# Autodesk Inventor assembly: BoxBeamDBAssembly
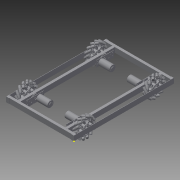
[picture p0: Inventor's stored thumbnail of the model, 180x180]
Saved by Autodesk Inventor 2015 (Build 190159000, 159)
## iProperties
Created: 2015-01-14
Part Number: BoxBeamDBAssembly
Document SubType Name: Assembly
Designer: chapale16
Author: chapale16
## Documents named in this file (13)
- \\lhssvr02\Homedirs\Robotics Club\CAD Model 2015\CDR prep\BoxBeamDBAssembly.iam
- \\lhssvr02\Homedirs\Robotics Club\CAD Model 2015\CDR prep\Frame front-back.ipt
- \\lhssvr02\Homedirs\Robotics Club\CAD Model 2015\CDR prep\Frame sides.ipt
- \\lhssvr02\Homedirs\Robotics Club\CAD Model 2015\Parts Folder\Wheels\Right Vex Mec Wheel.iam
- \\lhssvr02\Homedirs\Robotics Club\CAD Model 2015\Parts Folder\Gear Boxes\CIMple Box with motors.iam
- \\lhssvr02\Homedirs\Robotics Club\CAD Model 2015\CDR prep\Bumpers.ipt
- \\lhssvr02\Homedirs\Robotics Club\CAD Model 2015\GearBox Assembly_MIR.iam
- \\lhssvr02\Homedirs\Robotics Club\CAD Model 2015\Parts Folder\Wheels\Right Vex Mec Wheel_MIR.iam
- \\lhssvr02\Homedirs\Robotics Club\CAD Model 2015\GearBox Assembly_MIR_MIR.iam
- \\lhssvr02\Homedirs\Robotics Club\CAD Model 2015\Parts Folder\Wheels\Right Vex Mec Wheel_MIR1.iam
- \\lhssvr02\Homedirs\Robotics Club\CAD Model 2015\GearBox Assembly_MIR_MIR1.iam
- \\lhssvr02\Homedirs\Robotics Club\CAD Model 2015\Parts Folder\Wheels\Right Vex Mec Wheel_MIR_MIR.iam
- \\lhssvr02\Homedirs\Robotics Club\CAD Model 2015\GearBox Assembly_MIR_MIR_MIR.iam
## Components (18 placed, 12 different names)
1. Frame front-back:1 — Mate:3, Flush:5, Flush:6, Flush:7, Mate:4, Mate:5, Flush:8, Symmetry:1
2. Frame front-back:2 — Mate:1, Flush:1, Flush:2, Mate:2, Flush:3, Flush:4, Mate:6, Flush:9, Mate:7, Symmetry:1
3. Frame sides:1 — Mate:1, Flush:1, Flush:2, Mate:3, Flush:5, Flush:6, Mate:8, Mate:9, Mate:10, Symmetry:2
4. Frame sides:2 — Mate:2, Flush:3, Flush:4, Flush:7, Symmetry:2
5. Right Vex Mec Wheel:2 [sub-assembly] — Mate:10, Mate:11
6. CIMple Box with motors:1 [sub-assembly]
7. CIMple Box with motors:2 [sub-assembly]
8. CIMple Box with motors:3 [sub-assembly]
9. CIMple Box with motors:4 [sub-assembly]
10. Bumpers:1 — Mate:6, Flush:9, Mate:7
11. Bumpers:2 — Mate:4, Mate:5, Flush:8, Angle:1, Mate:11
12. GearBox Assembly_MIR:1 [sub-assembly] — Mate:8, Angle:1, Mate:9
13. Right Vex Mec Wheel_MIR:1 [sub-assembly]
14. GearBox Assembly_MIR_MIR:1 [sub-assembly]
15. Right Vex Mec Wheel_MIR1:1 [sub-assembly]
16. GearBox Assembly_MIR_MIR1:1 [sub-assembly]
17. Right Vex Mec Wheel_MIR_MIR:1 [sub-assembly]
18. GearBox Assembly_MIR_MIR_MIR:1 [sub-assembly]
## Relationships (23: Mate 11, Flush 9, Symmetry 2, Angle 1)
- Mate:1: Frame front-back:2 ↔ Frame sides:1
- Flush:1: Frame front-back:2 ↔ Frame sides:1
- Flush:2 (-88.9 mm): Frame front-back:2 ↔ Frame sides:1
- Mate:2: Frame front-back:2 ↔ Frame sides:2
- Flush:3: Frame front-back:2 ↔ Frame sides:2
- Flush:4 (88.9 mm): Frame front-back:2 ↔ Frame sides:2
- Mate:3: Frame front-back:1 ↔ Frame sides:1
- Flush:5: Frame front-back:1 ↔ Frame sides:1
- Flush:6 (-88.9 mm): Frame front-back:1 ↔ Frame sides:1
- Flush:7: Frame front-back:1 ↔ Frame sides:2
- Mate:4: Frame front-back:1 ↔ Bumpers:2
- Mate:5: Frame front-back:1 ↔ Bumpers:2
- Flush:8: Frame front-back:1 ↔ Bumpers:2
- Mate:6: Frame front-back:2 ↔ Bumpers:1
- Flush:9: Frame front-back:2 ↔ Bumpers:1
- Mate:7: Frame front-back:2 ↔ Bumpers:1
- Mate:8: Frame sides:1 ↔ GearBox Assembly_MIR:1
- Angle:1 (0 deg): Bumpers:2 ↔ GearBox Assembly_MIR:1
- Mate:9 (21.59 mm): Frame sides:1 ↔ GearBox Assembly_MIR:1
- Mate:10: Frame sides:1 ↔ Right Vex Mec Wheel:2
- Mate:11 (22.86 mm): Right Vex Mec Wheel:2 ↔ Bumpers:2
- Symmetry:1: Frame front-back:1 ↔ Frame front-back:2
- Symmetry:2: Frame sides:1 ↔ Frame sides:2
